# Autodesk Inventor assembly: Front Hub Carrier L
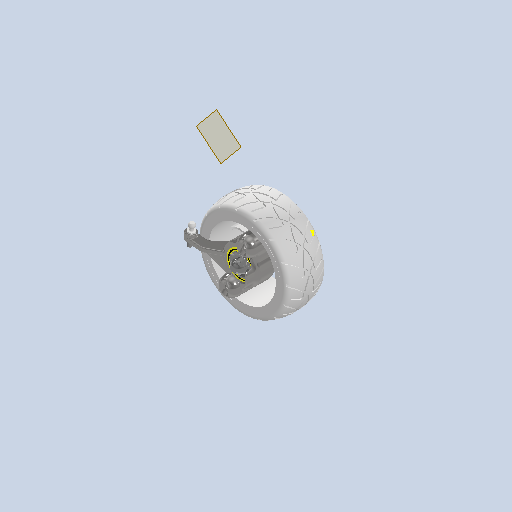
[picture p0: Inventor's stored thumbnail of the model, 512x512]
Saved by Autodesk Inventor 2024 (Build 280153000, 153)
## iProperties
Created: 2023-07-06
Part Number: Front Hub Carrier L
Document SubType Name: Assembly
Designer: birud
Author: birud
## Documents named in this file (14)
- C:\Users\_Astitva_Aryan_\Downloads\ES101_Components_Group5\Components_derived\Front Hub Carrier L.iam
- C:\Users\_Astitva_Aryan_\Downloads\ES101_Components_Group5\Components_derived\Front hub carrier L.ipt
- C:\Users\_Astitva_Aryan_\Downloads\ES101_Components_Group5\Components_derived\Pillow Ball Retainer-1.ipt
- C:\Users\_Astitva_Aryan_\Downloads\ES101_Components_Group5\Components_derived\Pillow Ball Bushing.ipt
- C:\Users\_Astitva_Aryan_\Downloads\ES101_Components_Group5\Components_derived\rear hub bearing.ipt
- C:\Users\_Astitva_Aryan_\Downloads\ES101_Components_Group5\Components_derived\front axle.ipt
- C:\Users\_Astitva_Aryan_\Downloads\ES101_Components_Group5\Components_derived\front hub bearing.ipt
- C:\Users\_Astitva_Aryan_\Downloads\ES101_Components_Group5\Components_derived\Ball Stud.ipt
- C:\Users\_Astitva_Aryan_\Downloads\ES101_Components_Group5\Components_derived\HexDrive.ipt
- C:\Users\_Astitva_Aryan_\Downloads\ES101_Components_Group5\Components_derived\hex axle pin.ipt
- C:\Users\_Astitva_Aryan_\Downloads\ES101_Components_Group5\Components_derived\hex retaining o-ring.ipt
- C:\Users\_Astitva_Aryan_\Downloads\ES101_Components_Group5\Components_derived\Wheel.ipt
- C:\Users\_Astitva_Aryan_\Downloads\ES101_Components_Group5\Components_derived\Tire.ipt
- C:\Users\_Astitva_Aryan_\Downloads\ES101_Components_Group5\Components_derived\ansi.ipt
## Components (15 placed, 13 different names)
1. Front hub carrier L:1 — Mate:1, Flush:1, Mate:3, Flush:2, Mate:5, Flush:3, Mate:6, Mate:8, Mate:9, Insert:1, Flush:4
2. Pillow Ball Retainer-1:1 — Mate:1, Flush:1, Mate:2, Rotational:1
3. Pillow Ball Bushing:1 — Mate:2, Rotational:1
4. Pillow Ball Retainer-1:2 — Mate:3, Flush:2, Mate:4, Rotational:2
5. Pillow Ball Bushing:2 — Mate:4, Rotational:2
6. rear hub bearing:1 — Mate:5, Flush:3
7. front axle:1 — Mate:6, Flush:4, Mate:14, Mate:15, Mate:18, Mate:20
8. front hub bearing:1 — Mate:8, Mate:9
9. Ball Stud:1 — Insert:1
10. HexDrive:1 — Mate:10, Mate:11, Mate:12, Mate:13, Mate:14, Mate:19
11. hex axle pin:1 — Mate:10, Mate:11, Mate:15
12. hex retaining o-ring:1 — Mate:12, Flush:5
13. Wheel:1 — Mate:16, Mate:17, Mate:18, Mate:19, Angle:1, Mate:21
14. Tire:1 — Mate:16, Mate:17, Angle:1
15. ansi:1 — Mate:20, Mate:21
## Relationships (29: Mate 20, Flush 5, RevoluteJoint 2, Insert 1, Angle 1)
- Mate:1: Front hub carrier L:1 ↔ Pillow Ball Retainer-1:1
- Flush:1 (38.1 mm): Front hub carrier L:1 ↔ Pillow Ball Retainer-1:1
- Mate:2: Pillow Ball Retainer-1:1 ↔ Pillow Ball Bushing:1
- Rotational:1 [RevoluteJoint]: Pillow Ball Retainer-1:1 ↔ Pillow Ball Bushing:1
- Mate:3: Front hub carrier L:1 ↔ Pillow Ball Retainer-1:2
- Flush:2 (38.1 mm): Front hub carrier L:1 ↔ Pillow Ball Retainer-1:2
- Mate:4: Pillow Ball Retainer-1:2 ↔ Pillow Ball Bushing:2
- Rotational:2 [RevoluteJoint]: Pillow Ball Retainer-1:2 ↔ Pillow Ball Bushing:2
- Mate:5: Front hub carrier L:1 ↔ rear hub bearing:1
- Flush:3: Front hub carrier L:1 ↔ rear hub bearing:1
- Mate:6: Front hub carrier L:1 ↔ front axle:1
- Mate:8: Front hub carrier L:1 ↔ front hub bearing:1
- Mate:9: Front hub carrier L:1 ↔ front hub bearing:1
- Insert:1: Front hub carrier L:1 ↔ Ball Stud:1
- Mate:10: HexDrive:1 ↔ hex axle pin:1
- Mate:11: HexDrive:1 ↔ hex axle pin:1
- Flush:4 (-142.875 mm): Front hub carrier L:1 ↔ front axle:1
- Mate:12: HexDrive:1 ↔ hex retaining o-ring:1
- Flush:5 (8.001 mm): hex retaining o-ring:1
- Mate:13: HexDrive:1
- Mate:14: front axle:1 ↔ HexDrive:1
- Mate:15: front axle:1 ↔ hex axle pin:1
- Mate:16: Wheel:1 ↔ Tire:1
- Mate:17: Wheel:1 ↔ Tire:1
- Mate:18: front axle:1 ↔ Wheel:1
- Mate:19: HexDrive:1 ↔ Wheel:1
- Angle:1 (0 deg): Wheel:1 ↔ Tire:1
- Mate:20: front axle:1 ↔ ansi:1
- Mate:21: Wheel:1 ↔ ansi:1
